# Autodesk Inventor assembly: КВ33.044.000
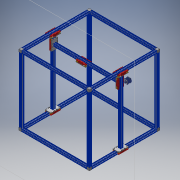
[picture p0: Inventor's stored thumbnail of the model, 180x180]
Saved by Autodesk Inventor 2019 (Build 230136000, 136)
## iProperties
Created: 2019-07-15
Part Number: КВ33.044.000
Material: Типовые
Document SubType Name: Assembly
Designer: Петров Иван
Description: Сортирующая ячейка
Author: Петров Иван
## Documents named in this file (6)
- C:\Users\user\Documents\Kvantoriada2019\optimal_gripper\hardware\КВ33.044.000 - Сортирующая ячейка.iam
- C:\Users\user\Documents\Kvantoriada2019\optimal_gripper\hardware\Стандартные изделия\Профиль станочный 30x30x740.ipt
- C:\Users\user\Documents\Kvantoriada2019\optimal_gripper\hardware\Стандартные изделия\Угол соединительный 30х30х30.ipt
- C:\Users\user\Documents\Kvantoriada2019\optimal_gripper\hardware\КВ33.044.200 - Каретка оси Х.iam
- C:\Users\user\Documents\Kvantoriada2019\optimal_gripper\hardware\Стандартные изделия\Профиль станочный 30x30x728.ipt
- C:\Users\user\Documents\Kvantoriada2019\optimal_gripper\hardware\Стандартные изделия\Шаговый двигатель Nema 17.ipt
## Components (31 placed, 5 different names)
1. Профиль станочный 30x30x740:1 — Заподлицо:9, Заподлицо:10, Совмещение:4, Заподлицо:12, Совмещение:9, Заподлицо:17
2. Профиль станочный 30x30x740:2 — Совмещение:3, Заподлицо:2, Заподлицо:3
3. Профиль станочный 30x30x740:3 — Совмещение:1, Заподлицо:1, Заподлицо:5, Заподлицо:6, Заподлицо:8, Совмещение:5
4. Профиль станочный 30x30x740:4 — Заподлицо:14, Совмещение:7, Заподлицо:16, Заподлицо:18, Заподлицо:19, Совмещение:10
5. Угол соединительный 30х30х30:1 — Совмещение:1, Совмещение:2, Совмещение:3, Заподлицо:1, Заподлицо:2, Заподлицо:3, Заподлицо:4, Заподлицо:5, Заподлицо:38
6. Угол соединительный 30х30х30:2 — Заподлицо:18, Заподлицо:19, Совмещение:10, Совмещение:11, Заподлицо:20, Заподлицо:21
7. Угол соединительный 30х30х30:3 — Заподлицо:6, Заподлицо:7, Заподлицо:8, Заподлицо:9, Заподлицо:10, Совмещение:4, Заподлицо:11, Совмещение:5, Совмещение:6
8. Угол соединительный 30х30х30:4 — Заподлицо:12, Заподлицо:13, Заподлицо:14, Заподлицо:15, Совмещение:7, Совмещение:8, Заподлицо:16, Совмещение:9, Заподлицо:17
9. Профиль станочный 30x30x740:9 — Заподлицо:7, Заподлицо:11, Совмещение:6, Совмещение:19, Заподлицо:36, Заподлицо:37, Совмещение:58, Касательность:20, Касательность:21
10. Профиль станочный 30x30x740:10 — Заподлицо:13, Заподлицо:15, Совмещение:8
11. Профиль станочный 30x30x740:11 — Совмещение:11, Заподлицо:20, Заподлицо:21
12. Профиль станочный 30x30x740:12 — Совмещение:2, Заподлицо:4, Заподлицо:38, Совмещение:51, Касательность:18, Касательность:19
13. Профиль станочный 30x30x740:15
14. Профиль станочный 30x30x740:16
15. Профиль станочный 30x30x740:17
16. Профиль станочный 30x30x740:18
17. Угол соединительный 30х30х30:5
18. Угол соединительный 30х30х30:6
19. Угол соединительный 30х30х30:7 — Совмещение:19, Заподлицо:36, Заподлицо:37
20. Угол соединительный 30х30х30:8
21. КВ33.044.200 - Каретка оси Х:6 [sub-assembly] — Совмещение:42, Совмещение:59, Совмещение:60, Совмещение:64, Касательность:22, Касательность:23
22. КВ33.044.200 - Каретка оси Х:7 [sub-assembly] — Совмещение:61, Совмещение:62, Совмещение:63, Касательность:24, Совмещение:65
23. Профиль станочный 30x30x728:4 — Совмещение:41, Касательность:16, Касательность:17, Совмещение:42, Совмещение:59, Совмещение:60, Совмещение:61, Совмещение:62, Совмещение:63
24. КВ33.044.200 - Каретка оси Х:8 [sub-assembly] — Совмещение:41, Касательность:16, Касательность:17
25. КВ33.044.200 - Каретка оси Х:9 [sub-assembly] — Совмещение:44, Совмещение:45, Совмещение:46, Совмещение:51, Касательность:18, Касательность:19
26. КВ33.044.200 - Каретка оси Х:10 [sub-assembly] — Совмещение:48, Совмещение:49, Совмещение:50
27. Профиль станочный 30x30x728:5 — Совмещение:44, Совмещение:45, Совмещение:46, Совмещение:48, Совмещение:49, Совмещение:50, Совмещение:64, Касательность:22, Касательность:23
28. КВ33.044.200 - Каретка оси Х:11 [sub-assembly] — Совмещение:58, Касательность:20, Касательность:21
29. КВ33.044.200 - Каретка оси Х:12 [sub-assembly]
30. Профиль станочный 30x30x728:6 — Касательность:24
31. Шаговый двигатель Nema 17:1 — Совмещение:65
## Relationships (89: Mate 42, Flush 38, Tangent 9)
- Совмещение:1 [Mate]: Профиль станочный 30x30x740:3 ↔ Угол соединительный 30х30х30:1
- Совмещение:2 [Mate]: Угол соединительный 30х30х30:1 ↔ Профиль станочный 30x30x740:12
- Совмещение:3 [Mate]: Профиль станочный 30x30x740:2 ↔ Угол соединительный 30х30х30:1
- Заподлицо:1 [Flush]: Профиль станочный 30x30x740:3 ↔ Угол соединительный 30х30х30:1
- Заподлицо:2 [Flush]: Профиль станочный 30x30x740:2 ↔ Угол соединительный 30х30х30:1
- Заподлицо:3 [Flush]: Профиль станочный 30x30x740:2 ↔ Угол соединительный 30х30х30:1
- Заподлицо:4 [Flush]: Угол соединительный 30х30х30:1 ↔ Профиль станочный 30x30x740:12
- Заподлицо:5 [Flush]: Профиль станочный 30x30x740:3 ↔ Угол соединительный 30х30х30:1
- Заподлицо:6 [Flush]: Профиль станочный 30x30x740:3 ↔ Угол соединительный 30х30х30:3
- Заподлицо:7 [Flush]: Угол соединительный 30х30х30:3 ↔ Профиль станочный 30x30x740:9
- Заподлицо:8 [Flush]: Профиль станочный 30x30x740:3 ↔ Угол соединительный 30х30х30:3
- Заподлицо:9 [Flush]: Профиль станочный 30x30x740:1 ↔ Угол соединительный 30х30х30:3
- Заподлицо:10 [Flush]: Профиль станочный 30x30x740:1 ↔ Угол соединительный 30х30х30:3
- Совмещение:4 [Mate]: Профиль станочный 30x30x740:1 ↔ Угол соединительный 30х30х30:3
- Заподлицо:11 [Flush]: Угол соединительный 30х30х30:3 ↔ Профиль станочный 30x30x740:9
- Совмещение:5 [Mate]: Профиль станочный 30x30x740:3 ↔ Угол соединительный 30х30х30:3
- Совмещение:6 [Mate]: Угол соединительный 30х30х30:3 ↔ Профиль станочный 30x30x740:9
- Заподлицо:12 [Flush]: Профиль станочный 30x30x740:1 ↔ Угол соединительный 30х30х30:4
- Заподлицо:13 [Flush]: Угол соединительный 30х30х30:4 ↔ Профиль станочный 30x30x740:10
- Заподлицо:14 [Flush]: Профиль станочный 30x30x740:4 ↔ Угол соединительный 30х30х30:4
- Заподлицо:15 [Flush]: Угол соединительный 30х30х30:4 ↔ Профиль станочный 30x30x740:10
- Совмещение:7 [Mate]: Профиль станочный 30x30x740:4 ↔ Угол соединительный 30х30х30:4
- Совмещение:8 [Mate]: Угол соединительный 30х30х30:4 ↔ Профиль станочный 30x30x740:10
- Заподлицо:16 [Flush]: Профиль станочный 30x30x740:4 ↔ Угол соединительный 30х30х30:4
- Совмещение:9 [Mate]: Профиль станочный 30x30x740:1 ↔ Угол соединительный 30х30х30:4
- Заподлицо:17 [Flush]: Профиль станочный 30x30x740:1 ↔ Угол соединительный 30х30х30:4
- Заподлицо:18 [Flush]: Профиль станочный 30x30x740:4 ↔ Угол соединительный 30х30х30:2
- Заподлицо:19 [Flush]: Профиль станочный 30x30x740:4 ↔ Угол соединительный 30х30х30:2
- Совмещение:10 [Mate]: Профиль станочный 30x30x740:4 ↔ Угол соединительный 30х30х30:2
- Совмещение:11 [Mate]: Угол соединительный 30х30х30:2 ↔ Профиль станочный 30x30x740:11
- Заподлицо:20 [Flush]: Угол соединительный 30х30х30:2 ↔ Профиль станочный 30x30x740:11
- Заподлицо:21 [Flush]: Угол соединительный 30х30х30:2 ↔ Профиль станочный 30x30x740:11
- [Mate]: Профиль станочный 30x30x740:17 ↔ Угол соединительный 30х30х30:5
- [Mate]: Профиль станочный 30x30x740:16 ↔ Угол соединительный 30х30х30:5
- [Flush]: Профиль станочный 30x30x740:17 ↔ Угол соединительный 30х30х30:5
- [Flush]: Профиль станочный 30x30x740:16 ↔ Угол соединительный 30х30х30:5
- [Flush]: Профиль станочный 30x30x740:16 ↔ Угол соединительный 30х30х30:5
- [Flush]: Профиль станочный 30x30x740:17 ↔ Угол соединительный 30х30х30:5
- [Flush]: Профиль станочный 30x30x740:17 ↔ Угол соединительный 30х30х30:7
- [Flush]: Профиль станочный 30x30x740:17 ↔ Угол соединительный 30х30х30:7
- [Flush]: Профиль станочный 30x30x740:15 ↔ Угол соединительный 30х30х30:7
- [Flush]: Профиль станочный 30x30x740:15 ↔ Угол соединительный 30х30х30:7
- [Mate]: Профиль станочный 30x30x740:15 ↔ Угол соединительный 30х30х30:7
- [Mate]: Профиль станочный 30x30x740:17 ↔ Угол соединительный 30х30х30:7
- [Flush]: Профиль станочный 30x30x740:15 ↔ Угол соединительный 30х30х30:8
- [Flush]: Профиль станочный 30x30x740:18 ↔ Угол соединительный 30х30х30:8
- [Mate]: Профиль станочный 30x30x740:18 ↔ Угол соединительный 30х30х30:8
- [Flush]: Профиль станочный 30x30x740:18 ↔ Угол соединительный 30х30х30:8
- [Mate]: Профиль станочный 30x30x740:15 ↔ Угол соединительный 30х30х30:8
- [Flush]: Профиль станочный 30x30x740:15 ↔ Угол соединительный 30х30х30:8
- [Flush]: Профиль станочный 30x30x740:18 ↔ Угол соединительный 30х30х30:6
- [Flush]: Профиль станочный 30x30x740:18 ↔ Угол соединительный 30х30х30:6
- [Mate]: Профиль станочный 30x30x740:18 ↔ Угол соединительный 30х30х30:6
- Совмещение:19 [Mate]: Профиль станочный 30x30x740:9 ↔ Угол соединительный 30х30х30:7
- Заподлицо:36 [Flush]: Профиль станочный 30x30x740:9 ↔ Угол соединительный 30х30х30:7
- Заподлицо:37 [Flush]: Профиль станочный 30x30x740:9 ↔ Угол соединительный 30х30х30:7
- Заподлицо:38 [Flush]: Угол соединительный 30х30х30:1 ↔ Профиль станочный 30x30x740:12
- Совмещение:41 [Mate]: Профиль станочный 30x30x728:4 ↔ КВ33.044.200 - Каретка оси Х:8
- Касательность:16 [Tangent]: Профиль станочный 30x30x728:4 ↔ КВ33.044.200 - Каретка оси Х:8
- Касательность:17 [Tangent]: Профиль станочный 30x30x728:4 ↔ КВ33.044.200 - Каретка оси Х:8
- Совмещение:42 [Mate]: КВ33.044.200 - Каретка оси Х:6 ↔ Профиль станочный 30x30x728:4
- Совмещение:44 [Mate]: КВ33.044.200 - Каретка оси Х:9 ↔ Профиль станочный 30x30x728:5
- Совмещение:45 [Mate]: КВ33.044.200 - Каретка оси Х:9 ↔ Профиль станочный 30x30x728:5
- Совмещение:46 [Mate]: КВ33.044.200 - Каретка оси Х:9 ↔ Профиль станочный 30x30x728:5
- Совмещение:48 [Mate]: КВ33.044.200 - Каретка оси Х:10 ↔ Профиль станочный 30x30x728:5
- Совмещение:49 [Mate]: КВ33.044.200 - Каретка оси Х:10 ↔ Профиль станочный 30x30x728:5
- Совмещение:50 [Mate]: КВ33.044.200 - Каретка оси Х:10 ↔ Профиль станочный 30x30x728:5
- Совмещение:51 [Mate]: Профиль станочный 30x30x740:12 ↔ КВ33.044.200 - Каретка оси Х:9
- Касательность:18 [Tangent]: Профиль станочный 30x30x740:12 ↔ КВ33.044.200 - Каретка оси Х:9
- Касательность:19 [Tangent]: Профиль станочный 30x30x740:12 ↔ КВ33.044.200 - Каретка оси Х:9
- [Mate]: КВ33.044.200 - Каретка оси Х:11 ↔ Профиль станочный 30x30x728:6
- [Mate]: КВ33.044.200 - Каретка оси Х:11 ↔ Профиль станочный 30x30x728:6
- [Mate]: КВ33.044.200 - Каретка оси Х:11 ↔ Профиль станочный 30x30x728:6
- [Mate]: КВ33.044.200 - Каретка оси Х:12 ↔ Профиль станочный 30x30x728:6
- [Mate]: КВ33.044.200 - Каретка оси Х:12 ↔ Профиль станочный 30x30x728:6
- [Mate]: КВ33.044.200 - Каретка оси Х:12 ↔ Профиль станочный 30x30x728:6
- Совмещение:58 [Mate]: Профиль станочный 30x30x740:9 ↔ КВ33.044.200 - Каретка оси Х:11
- Касательность:20 [Tangent]: Профиль станочный 30x30x740:9 ↔ КВ33.044.200 - Каретка оси Х:11
- Касательность:21 [Tangent]: Профиль станочный 30x30x740:9 ↔ КВ33.044.200 - Каретка оси Х:11
- Совмещение:59 [Mate]: КВ33.044.200 - Каретка оси Х:6 ↔ Профиль станочный 30x30x728:4
- Совмещение:60 [Mate]: КВ33.044.200 - Каретка оси Х:6 ↔ Профиль станочный 30x30x728:4
- Совмещение:61 [Mate]: КВ33.044.200 - Каретка оси Х:7 ↔ Профиль станочный 30x30x728:4
- Совмещение:62 [Mate]: КВ33.044.200 - Каретка оси Х:7 ↔ Профиль станочный 30x30x728:4
- Совмещение:63 [Mate]: КВ33.044.200 - Каретка оси Х:7 ↔ Профиль станочный 30x30x728:4
- Совмещение:64 [Mate]: КВ33.044.200 - Каретка оси Х:6 ↔ Профиль станочный 30x30x728:5
- Касательность:22 [Tangent]: КВ33.044.200 - Каретка оси Х:6 ↔ Профиль станочный 30x30x728:5
- Касательность:23 [Tangent]: КВ33.044.200 - Каретка оси Х:6 ↔ Профиль станочный 30x30x728:5
- Касательность:24 [Tangent]: КВ33.044.200 - Каретка оси Х:7 ↔ Профиль станочный 30x30x728:6
- Совмещение:65 [Mate]: КВ33.044.200 - Каретка оси Х:7 ↔ Шаговый двигатель Nema 17:1
## Named parameters: d91_d80 = 0 mm, d92_d82 = 0 mm, d93_d83 = 0 mm, d94_d84 = 0 mm, d95_d85 = 0 mm, d96_d86 = 0 mm, d97_d87 = 0 mm, d98_d66 = 0 mm, d99_d67 = 0 mm, d100_d69 = 0 mm, d101_d70 = 0 mm, d102_d71 = 0 mm, d103_d72 = 0 mm, d104_d74 = 0 mm, d105_d76 = 0 mm, d106_d78 = 0 mm, d107_d59 = 0 mm, d108_d61 = 0 mm, d109_d62 = 0 mm, d110_d63 = 0 mm, d111_d64 = 0 mm, d201_d189 = 0 mm, d202_d190 = 0 mm, d203_d191 = 0 mm, d204_d195 = 0 mm, d205_d196 = 0 mm, d206_d197 = 0 mm
